# Autodesk Inventor assembly: Breaker
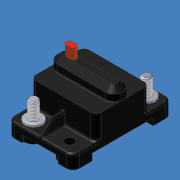
[picture p0: Inventor's stored thumbnail of the model, 180x180]
Saved by Autodesk Inventor 2013 (Build 170138000, 138)
## iProperties
Shininess: 64.0
Angle Display Precision: 2
Document Length Units: 11272
Document Angle Units: 11279
Document Time Units: 11290
Document Mass Units: 11286
Document Length Units Precision: 3
Document Angle Units Precision: 2
Created: 2004-01-20
Part Number: Breaker
Document SubType Name: Assembly
Designer: t8558es
Density: 0.0
Volumn: 0.0
Area: 0.0
PropertySet Name: Model Information
Control State: 0
Master: False
Checked Out: False
Author: t8558es
## Documents named in this file (3)
- C:\Users\carneeki\Google Drive\Robotics\FRC 2013\FRC2013 - LDU\Kiwi Robot\Imported Components\ELEC\Breaker\Breaker.iam
- C:\Users\carneeki\Google Drive\Robotics\FRC 2013\FRC2013 - LDU\Kiwi Robot\Imported Components\ELEC\Breaker\Breaker Body.ipt
- C:\Users\carneeki\Google Drive\Robotics\FRC 2013\FRC2013 - LDU\Kiwi Robot\Imported Components\ELEC\Breaker\Breaker Post.ipt
## Components (3 placed, 2 different names)
1. Breaker Body:1 — Mate:1, Mate:2, Mate:3, Mate:4
2. Breaker Post:1 — Mate:1, Mate:2
3. Breaker Post:2 — Mate:3, Mate:4
## Relationships (4: Mate 4)
- Mate:1: Breaker Body:1 ↔ Breaker Post:1
- Mate:2: Breaker Body:1 ↔ Breaker Post:1
- Mate:3: Breaker Body:1 ↔ Breaker Post:2
- Mate:4: Breaker Body:1 ↔ Breaker Post:2
